# Autodesk Inventor assembly: ajAsm
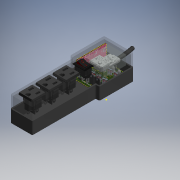
[picture p0: Inventor's stored thumbnail of the model, 180x180]
Saved by Autodesk Inventor 2018 (Build 220112000, 112)
## iProperties
Created: 2018-02-17
Part Number: ajAsm
Document SubType Name: Assembly
Designer: artur
Author: artur
## Documents named in this file (9)
- C:\Users\artur\Documents\projects\smartPowerStrip\CAD\Mechanical\ajAsm.iam
- C:\Users\artur\Documents\projects\smartPowerStrip\CAD\Mechanical\ajBottom.ipt
- C:\Users\artur\Documents\projects\smartPowerStrip\CAD\Mechanical\ajTop.ipt
- C:\Users\artur\Documents\projects\smartPowerStrip\CAD\Mechanical\QUALTEK 738W-X201.ipt
- C:\Users\artur\Documents\projects\smartPowerStrip\CAD\Mechanical\dimmerModule.ipt
- C:\Users\artur\Documents\projects\smartPowerStrip\CAD\Mechanical\ESP8266_ThingDevBoard.ipt
- C:\Users\artur\Documents\projects\smartPowerStrip\CAD\Mechanical\AC2DC_real.iam
- C:\Users\artur\Documents\projects\smartPowerStrip\CAD\Mechanical\wire.ipt
- C:\Users\artur\Documents\projects\smartPowerStrip\CAD\Mechanical\powerRocker.ipt
## Components (10 placed, 8 different names)
1. ajBottom:1 — Mate:1, Flush:1, Mate:2, Mate:12, Mate:13, Mate:14, Mate:15, Mate:16, Mate:17, Mate:21, Mate:22
2. ajTop:1 — Mate:1, Flush:1, Mate:2, Mate:3, Mate:4, Mate:5, Mate:6, Mate:7, Mate:8, Mate:9, Mate:10, Mate:11, Flush:2, Mate:18, Mate:19, Mate:20
3. QUALTEK 738W-X201:1 — Mate:5, Mate:6, Mate:11
4. QUALTEK 738W-X201:2 — Mate:3, Mate:7, Mate:9
5. QUALTEK 738W-X201:3 — Mate:4, Mate:8, Mate:10
6. dimmerModule:1 — Mate:12, Mate:13, Mate:22
7. ESP8266_ThingDevBoard:1 — Mate:16, Mate:17, Mate:21
8. AC2DC_real:1 [sub-assembly] — Mate:14, Mate:15
9. wire:1 — Flush:2
10. powerRocker:1 — Mate:18, Mate:19, Mate:20
## Relationships (24: Mate 22, Flush 2)
- Mate:1: ajBottom:1 ↔ ajTop:1
- Flush:1: ajBottom:1 ↔ ajTop:1
- Mate:2: ajBottom:1 ↔ ajTop:1
- Mate:3: ajTop:1 ↔ QUALTEK 738W-X201:2
- Mate:4: ajTop:1 ↔ QUALTEK 738W-X201:3
- Mate:5: ajTop:1 ↔ QUALTEK 738W-X201:1
- Mate:6: ajTop:1 ↔ QUALTEK 738W-X201:1
- Mate:7: ajTop:1 ↔ QUALTEK 738W-X201:2
- Mate:8: ajTop:1 ↔ QUALTEK 738W-X201:3
- Mate:9 (4.572 mm): ajTop:1 ↔ QUALTEK 738W-X201:2
- Mate:10 (4.572 mm): ajTop:1 ↔ QUALTEK 738W-X201:3
- Mate:11 (4.572 mm): ajTop:1 ↔ QUALTEK 738W-X201:1
- Mate:12 (5.08 mm): ajBottom:1 ↔ dimmerModule:1
- Mate:13 (1.27 mm): ajBottom:1 ↔ dimmerModule:1
- Mate:14 (25.4 mm): ajBottom:1 ↔ AC2DC_real:1
- Mate:15 (2.54 mm): ajBottom:1 ↔ AC2DC_real:1
- Mate:16 (5.08 mm): ajBottom:1 ↔ ESP8266_ThingDevBoard:1
- Mate:17 (12.7 mm): ajBottom:1 ↔ ESP8266_ThingDevBoard:1
- Flush:2: ajTop:1 ↔ wire:1
- Mate:18: ajTop:1 ↔ powerRocker:1
- Mate:19: ajTop:1 ↔ powerRocker:1
- Mate:20: ajTop:1 ↔ powerRocker:1
- Mate:21 (2.54 mm): ajBottom:1 ↔ ESP8266_ThingDevBoard:1
- Mate:22 (1.27 mm): ajBottom:1 ↔ dimmerModule:1
